# Autodesk Inventor assembly: wafel_rev2
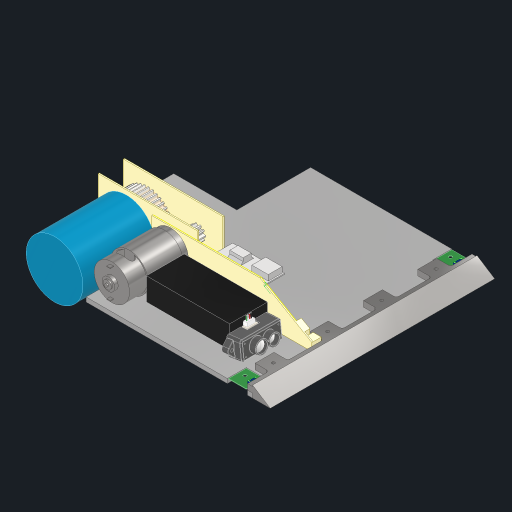
[picture p0: Inventor's stored thumbnail of the model, 512x512]
Saved by Autodesk Inventor 2023 (Build 270158000, 158)
## iProperties
Created: 2024-04-29
Part Number: wafel_rev2
Document SubType Name: Assembly
Designer: szymo
Mass: 1003.76 g
Surface Area: 2108.57 cm^2
Volume: 502.217 cm^3
Density: 1.99865 g/cm^3
Author: szymo
## iProperties of the stored document TFMINI_S_UART.ipt
Created: 2023-12-04
Part Number: TFMINI S UART
Material: Generic
Description: STEP AP214
Document SubType Name: Modeling
Designer: mateu
Density: 1 g/cm^3
Appearance: Default
Mass: 6.04913 g
Surface Area: 27.6076 cm^2
Volume: 6.04913 cm^3
Sending System: SolidWorks 2016
Preprocessor: SwSTEP 2.0
Title: TFMINI S UART.STEP
Author: USER
Revision Number: ANY
## Documents named in this file (23)
- D:\roboilo\robots\codename wafel - australia\3d_parts\rev3\wafel_rev3.iam
- D:\roboilo\robots\codename wafel - australia\3d_parts\rev3\plog.ipt
- D:\roboilo\robots\codename wafel - australia\3d_parts\rev3\smolgear_shaft.ipt
- D:\roboilo\robots\codename wafel - australia\3d_parts\rev3\stack.iam
- D:\roboilo\robots\codename wafel - australia\3d_parts\rev3\Switch.ipt
- D:\roboilo\robots\codename wafel - australia\3d_parts\rev3\wheel_axle.iam
- D:\roboilo\robots\codename wafel - australia\3d_parts\rev3\KTIR-Board.ipt
- D:\roboilo\robots\codename wafel - australia\3d_parts\rev3\lipo3s650.ipt
- D:\roboilo\robots\codename wafel - australia\3d_parts\rev3\Design Accelerator\smolGear.iam
- D:\roboilo\robots\codename wafel - australia\3d_parts\rev3\motor_w_gear.iam
- D:\roboilo\robots\codename wafel - australia\3d_parts\rev3\base.ipt
- D:\roboilo\robots\codename wafel - australia\3d_parts\rev3\wheel.ipt
- D:\roboilo\robots\codename wafel - australia\3d_parts\rev3\interface_board.ipt
- **D:\roboilo\robots\codename wafel - australia\3d_parts\rev3\wafel_rev3.iam*LocalDocs*xAaaaqfaaAaaaaaaaAaaaqmipFc*TFMINI_S_UART.ipt
- D:\roboilo\robots\codename wafel - australia\3d_parts\rev3\lipo2s450mah.ipt
- D:\roboilo\robots\codename wafel - australia\3d_parts\rev3\right_gear_holder.ipt
- D:\roboilo\robots\codename wafel - australia\3d_parts\rev3\right_gear_outerhold.ipt
- D:\roboilo\robots\codename wafel - australia\3d_parts\rev3\right_hold.ipt
- D:\roboilo\robots\codename wafel - australia\3d_parts\rev3\right_gear_holder_MIR.ipt
- D:\roboilo\robots\codename wafel - australia\3d_parts\rev3\right_gear_outerhold_MIR.ipt
- D:\roboilo\robots\codename wafel - australia\3d_parts\rev3\right_hold_MIR.ipt
- D:\roboilo\robots\codename wafel - australia\3d_parts\rev3\128x32-OLED.ipt
- D:\roboilo\robots\codename wafel - australia\3d_parts\rev3\TFMINI_S_UART.ipt
## Components (29 placed, 21 different names)
1. base:1 — Mate:1, Flush:1, Mate:3, Mate:4, Flush:2, Mate:5, Mate:6, Flush:3, Mate:8, Angle:1, Mate:9, Angle:2, Tangent:1, Tangent:2, Mate:12, Mate:13, Mate:16, Flush:8, Flush:9, Tangent:7, Tangent:8, Tangent:9, Tangent:10, Angle:7, Angle:8, Flush:14, Flush:16, Flush:17, Flush:18, Flush:19
2. plog:1 — Mate:2, Angle:3, Angle:4, Angle:5, Angle:6, Mate:14, Mate:15, Flush:20
3. right_gear_holder:1 — Flush:14, Flush:15
4. right_gear_outerhold:1 — Flush:16, Flush:17
5. right_hold:1 — Flush:18, Flush:19, Flush:20, Mate:25, Flush:21, Mate:26
6. right_gear_holder_MIR:1
7. right_gear_outerhold_MIR:1
8. right_hold_MIR:1 — Mate:27, Mate:28, Flush:22, Mate:29, Mate:30
9. wheel_axle:1 [sub-assembly] — Mate:8, Angle:1, Tangent:2, Flush:6, Tangent:3, Mate:17, Mate:19, Mate:21, Flush:12
10. smolGear:1 [sub-assembly] — Flush:6, Tangent:3, Tangent:4, Flush:7, Mate:23
11. wheel:1 — Mate:19, Mate:21
12. motor_w_gear:1 [sub-assembly] — Tangent:4, Flush:7, Tangent:7, Tangent:9, Angle:7
13. motor_w_gear:2 [sub-assembly] — Tangent:6, Flush:11, Tangent:8, Tangent:10, Angle:8
14. wheel_axle:2 [sub-assembly] — Mate:9, Angle:2, Tangent:1, Mate:18, Tangent:5, Flush:10, Mate:20, Mate:22, Flush:13
15. smolGear:2 [sub-assembly] — Tangent:5, Tangent:6, Flush:10, Flush:11, Mate:24
16. wheel:2 — Mate:20, Mate:22
17. smolgear_shaft:1 — Mate:23, Flush:12
18. smolgear_shaft:2 — Mate:24, Flush:13
19. stack:1 [sub-assembly] — Mate:1, Flush:1, Mate:2
20. Switch:1 — Mate:29, Mate:30, Mate:31
21. KTIR-Board:1 — Mate:3, Mate:4, Flush:2
22. KTIR-Board:2 — Mate:5, Mate:6, Flush:3
23. interface_board:1 — Mate:25, Flush:21, Mate:26
24. lipo2s450mah:1 — Mate:16, Flush:8, Flush:9, Mate:17, Mate:18, Flush:15
25. lipo3s650:1
26. lipo3s650:2
27. TFMINI_S_UART:1 — Mate:13, Angle:3, Angle:5, Mate:15
28. TFMINI_S_UART:2 — Mate:12, Angle:4, Angle:6, Mate:14
29. 128x32-OLED:1 — Mate:27, Mate:28, Flush:22, Mate:31
## Relationships (66: Mate 28, Flush 20, Tangent 10, Angle 8)
- Mate:1 (2 mm): base:1 ↔ stack:1
- Flush:1 (61.5 mm): base:1 ↔ stack:1
- Mate:2 (1 mm): plog:1 ↔ stack:1
- Mate:3 (0.5 mm): base:1 ↔ KTIR-Board:1
- Mate:4 (0.5 mm): base:1 ↔ KTIR-Board:1
- Flush:2: base:1 ↔ KTIR-Board:1
- Mate:5 (0.5 mm): base:1 ↔ KTIR-Board:2
- Mate:6 (0.5 mm): base:1 ↔ KTIR-Board:2
- Flush:3: base:1 ↔ KTIR-Board:2
- Mate:8 (-25 mm): base:1 ↔ wheel_axle:1
- Angle:1 (0 deg): base:1 ↔ wheel_axle:1
- Mate:9 (-25 mm): base:1 ↔ wheel_axle:2
- Angle:2 (0 deg): base:1 ↔ wheel_axle:2
- Tangent:1 (1 mm): base:1 ↔ wheel_axle:2
- Tangent:2 (1 mm): base:1 ↔ wheel_axle:1
- Mate:12: base:1 ↔ TFMINI_S_UART:2
- Mate:13: base:1 ↔ TFMINI_S_UART:1
- Angle:3 (-6.5 deg): plog:1 ↔ TFMINI_S_UART:1
- Angle:4 (6.5 deg): plog:1 ↔ TFMINI_S_UART:2
- Angle:5 (0 deg): plog:1 ↔ TFMINI_S_UART:1
- Angle:6 (0 deg): plog:1 ↔ TFMINI_S_UART:2
- Mate:14 (3.5 mm): plog:1 ↔ TFMINI_S_UART:2
- Mate:15 (3.5 mm): plog:1 ↔ TFMINI_S_UART:1
- Flush:6: wheel_axle:1 ↔ smolGear:1
- Tangent:3: wheel_axle:1 ↔ smolGear:1
- Tangent:4: smolGear:1 ↔ motor_w_gear:1
- Flush:7: smolGear:1 ↔ motor_w_gear:1
- Mate:16: base:1 ↔ lipo2s450mah:1
- Flush:8: base:1 ↔ lipo2s450mah:1
- Flush:9 (80.5 mm): base:1 ↔ lipo2s450mah:1
- Mate:17 (1 mm): wheel_axle:1 ↔ lipo2s450mah:1
- Mate:18 (1 mm): wheel_axle:2 ↔ lipo2s450mah:1
- Tangent:5: wheel_axle:2 ↔ smolGear:2
- Tangent:6: motor_w_gear:2 ↔ smolGear:2
- Flush:10: wheel_axle:2 ↔ smolGear:2
- Flush:11: motor_w_gear:2 ↔ smolGear:2
- Tangent:7: base:1 ↔ motor_w_gear:1
- Tangent:8: base:1 ↔ motor_w_gear:2
- Tangent:9: base:1 ↔ motor_w_gear:1
- Tangent:10: base:1 ↔ motor_w_gear:2
- Angle:7 (0 deg): base:1 ↔ motor_w_gear:1
- Angle:8 (0 deg): base:1 ↔ motor_w_gear:2
- Mate:19: wheel_axle:1 ↔ wheel:1
- Mate:20: wheel_axle:2 ↔ wheel:2
- Mate:21: wheel_axle:1 ↔ wheel:1
- Mate:22: wheel_axle:2 ↔ wheel:2
- Mate:23: smolGear:1 ↔ smolgear_shaft:1
- Flush:12: wheel_axle:1 ↔ smolgear_shaft:1
- Mate:24: smolGear:2 ↔ smolgear_shaft:2
- Flush:13: wheel_axle:2 ↔ smolgear_shaft:2
- Flush:14: base:1 ↔ right_gear_holder:1
- Flush:15: right_gear_holder:1 ↔ lipo2s450mah:1
- Flush:16: base:1 ↔ right_gear_outerhold:1
- Flush:17: base:1 ↔ right_gear_outerhold:1
- Flush:18: base:1 ↔ right_hold:1
- Flush:19: base:1 ↔ right_hold:1
- Flush:20: plog:1 ↔ right_hold:1
- Mate:25: right_hold:1 ↔ interface_board:1
- Flush:21 (2 mm): right_hold:1 ↔ interface_board:1
- Mate:26: right_hold:1 ↔ interface_board:1
- Mate:27 (-2 mm): right_hold_MIR:1 ↔ 128x32-OLED:1
- Mate:28: right_hold_MIR:1 ↔ 128x32-OLED:1
- Flush:22 (-3 mm): right_hold_MIR:1 ↔ 128x32-OLED:1
- Mate:29: right_hold_MIR:1 ↔ Switch:1
- Mate:30 (-4 mm): right_hold_MIR:1 ↔ Switch:1
- Mate:31 (1.2 mm): Switch:1 ↔ 128x32-OLED:1
